# Autodesk Inventor assembly: Herramienta Marcador
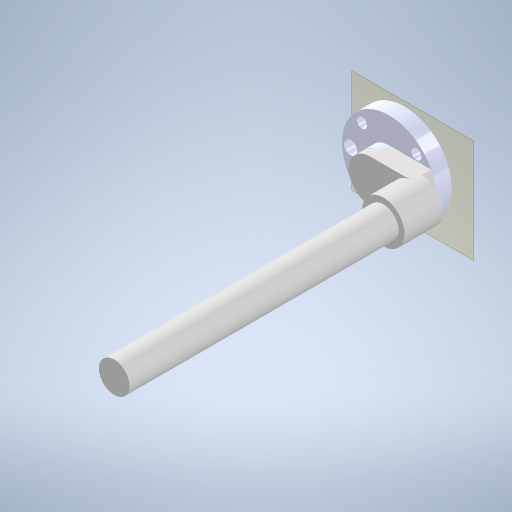
[picture p0: Inventor's stored thumbnail of the model, 512x512]
Saved by Autodesk Inventor 2023 (Build 270158000, 158)
## iProperties
Created: 2023-02-19
Part Number: Herramienta Marcador
Document SubType Name: Assembly
Designer: luisd
Author: luisd
## Documents named in this file (4)
- C:\Users\luisd\OneDrive\Documents\UNAL\Noveno Semestre\Robótica\Labs\Lab 1\Herramienta Marcador\Herramienta Marcador.iam
- C:\Users\luisd\OneDrive\Documents\UNAL\Noveno Semestre\Robótica\Labs\Lab 1\Herramienta Marcador\Herramienta Marcador Base.ipt
- C:\Users\luisd\OneDrive\Documents\UNAL\Noveno Semestre\Robótica\Labs\Lab 1\Herramienta Marcador\Herramienta Marcador Conector.ipt
- C:\Users\luisd\OneDrive\Documents\UNAL\Noveno Semestre\Robótica\Labs\Lab 1\Herramienta Marcador\Marcador.ipt
## Components (3 placed, 3 different names)
1. Herramienta Marcador Base:1 — Mate:1, Mate:2, Mate:4, Mate:7, Mate:8
2. Herramienta Marcador Conector:1 — Mate:1, Mate:2, Mate:4, Mate:5, Mate:6
3. Marcador:1 — Mate:5, Mate:6
## Relationships (7: Mate 7)
- Mate:1: Herramienta Marcador Base:1 ↔ Herramienta Marcador Conector:1
- Mate:2: Herramienta Marcador Base:1 ↔ Herramienta Marcador Conector:1
- Mate:4: Herramienta Marcador Base:1 ↔ Herramienta Marcador Conector:1
- Mate:5: Herramienta Marcador Conector:1 ↔ Marcador:1
- Mate:6: Herramienta Marcador Conector:1 ↔ Marcador:1
- Mate:7: Herramienta Marcador Base:1
- Mate:8: Herramienta Marcador Base:1
